# Autodesk Inventor assembly: złożenie przekładni
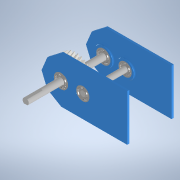
[picture p0: Inventor's stored thumbnail of the model, 180x180]
Saved by Autodesk Inventor 2021 (Build 250183000, 183)
## iProperties
Created: 2021-06-25
Part Number: złożenie przekładni
Document SubType Name: Assembly
Designer: Łukasz
Author: Łukasz
## Documents named in this file (8)
- E:\GITHUB_Czołg\Szybki-Czolg-antyRadziecki\złożenie przekładni.iam
- E:\GITHUB_Czołg\Szybki-Czolg-antyRadziecki\oś napędowa 12mm.ipt
- E:\GITHUB_Czołg\Szybki-Czolg-antyRadziecki\obudowa przekładni.ipt
- C:\Users\Łukasz\Documents\Inventor\Content Center Files\R2021\en-US\BS 292 (I)\BS 292 Part 1 - 6001 - 12 x 28 x 8.ipt
- E:\GITHUB_Czołg\Szybki-Czolg-antyRadziecki\oś 12 91mm.ipt
- E:\GITHUB_Czołg\Szybki-Czolg-antyRadziecki\koła zębate\Design Accelerator\Spur Gear11.ipt
- E:\GITHUB_Czołg\Szybki-Czolg-antyRadziecki\koła zębate\Design Accelerator\Spur Gear21.ipt
- C:\Users\Łukasz\Documents\Inventor\Content Center Files\R2021\en-US\BS 292 (I)\BS 292 Part 1 - 6000 - 10 x 26 x 8.ipt
## Components (9 placed, 7 different names)
1. oś napędowa 12mm:1 — Rotational:4, Rigid:2
2. obudowa przekładni:1 — Rotational:1, Rigid:1, Rotational:2, Rotational:3
3. BS 292: Part 1 (I) (Metric) 6000 - 10 x 26 x 8:2 — Rotational:3, Rotational:5
4. BS 292: Part 1 (I) (Metric) 6001 - 12 x 28 x 8:2 — Rotational:1
5. BS 292: Part 1 (I) (Metric) 6001 - 12 x 28 x 8:3 — Rotational:2, Rotational:4
6. BS 292: Part 1 (I) (Metric) 6000 - 10 x 26 x 8:1 — Rigid:1, Rotational:7
7. oś 12 91mm:1 — Rotational:5
8. Spur Gear1:1 — Rotational:7, Rotation:1
9. Spur Gear2:1 — Rotation:1, Rigid:2
## Relationships (9: RevoluteJoint 6, WeldJoint 2, RelateRotation 1)
- Rotational:1 [RevoluteJoint]: obudowa przekładni:1 ↔ BS 292: Part 1 (I) (Metric) 6001 - 12 x 28 x 8:2
- Rigid:1 [WeldJoint]: obudowa przekładni:1 ↔ BS 292: Part 1 (I) (Metric) 6000 - 10 x 26 x 8:1
- Rotational:2 [RevoluteJoint]: obudowa przekładni:1 ↔ BS 292: Part 1 (I) (Metric) 6001 - 12 x 28 x 8:3
- Rotational:3 [RevoluteJoint]: obudowa przekładni:1 ↔ BS 292: Part 1 (I) (Metric) 6000 - 10 x 26 x 8:2
- Rotational:4 [RevoluteJoint]: oś napędowa 12mm:1 ↔ BS 292: Part 1 (I) (Metric) 6001 - 12 x 28 x 8:3
- Rotational:5 [RevoluteJoint]: BS 292: Part 1 (I) (Metric) 6000 - 10 x 26 x 8:2 ↔ oś 12 91mm:1
- Rotational:7 [RevoluteJoint] (2 mm): BS 292: Part 1 (I) (Metric) 6000 - 10 x 26 x 8:1 ↔ Spur Gear1:1
- Rotation:1 [RelateRotation] (3 ul): Spur Gear1:1 ↔ Spur Gear2:1
- Rigid:2 [WeldJoint] (1 mm): oś napędowa 12mm:1 ↔ Spur Gear2:1
